# Autodesk Inventor assembly: Humidifier Assembly
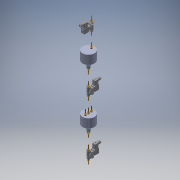
[picture p0: Inventor's stored thumbnail of the model, 180x180]
Saved by Autodesk Inventor 2018 (Build 220112000, 112)
## iProperties
Created: 2020-03-31
Part Number: Humidifier Assembly
Description: STEP AP214
Document SubType Name: Assembly
Designer: emile
Sending System: SolidWorks 2017
Preprocessor: SwSTEP 2.0
Title: Humidifier Assembly.STEP
Revision Number: ANY
## Documents named in this file (5)
- C:\Users\emile\OneDrive\Documents\GitHub\VentilatorCovid19\Respirator\MultiLine\Humidificator\Humidifier Assembly.iam
- C:\Users\emile\OneDrive\Documents\GitHub\VentilatorCovid19\Respirator\MultiLine\Humidificator\Humidifier Botom Funnel.ipt
- C:\Users\emile\OneDrive\Documents\GitHub\VentilatorCovid19\Respirator\MultiLine\SolenoidValve.iam
- C:\Users\emile\OneDrive\Documents\GitHub\VentilatorCovid19\Respirator\Peep\AirPressure\Brass Barbed Hose Fitting for Air and Water.ipt
- C:\Users\emile\OneDrive\Documents\GitHub\VentilatorCovid19\Respirator\MultiLine\Humidificator\HumidifierTopFunnel.ipt
## Components (11 placed, 4 different names)
1. Humidifier Botom Funnel_1 — Mate:1, Mate:2, Mate:11, Mate:12, Mate:15
2. Humidifier Botom Funnel_2 — Mate:5, Mate:6, Mate:7, Mate:8, Mate:9, Mate:10, Mate:13, Mate:14, Mate:15
3. SolenoidValve:1 [sub-assembly] — Mate:17, Angle:1, Mate:18, Mate:19, Flush:1
4. SolenoidValve:2 [sub-assembly] — Mate:20, Angle:2
5. Brass Barbed Hose Fitting for Air and Water:1 — Mate:1, Mate:2, Mate:16, Mate:20
6. Brass Barbed Hose Fitting for Air and Water:4 — Mate:6, Mate:9, Mate:18
7. Brass Barbed Hose Fitting for Air and Water:5 — Mate:5, Mate:8, Mate:16
8. Brass Barbed Hose Fitting for Air and Water:6 — Mate:7, Mate:10
9. Brass Barbed Hose Fitting for Air and Water:7 — Mate:13, Mate:14, Mate:21, Mate:22
10. Brass Barbed Hose Fitting for Air and Water:8 — Mate:11, Mate:12, Mate:17, Mate:19
11. SolenoidValve:3 [sub-assembly] — Mate:21, Mate:22, Flush:1
## Relationships (23: Mate 20, Angle 2, Flush 1)
- Mate:1: Humidifier Botom Funnel_1 ↔ Brass Barbed Hose Fitting for Air and Water:1
- Mate:2: Humidifier Botom Funnel_1 ↔ Brass Barbed Hose Fitting for Air and Water:1
- Mate:5: Humidifier Botom Funnel_2 ↔ Brass Barbed Hose Fitting for Air and Water:5
- Mate:6: Humidifier Botom Funnel_2 ↔ Brass Barbed Hose Fitting for Air and Water:4
- Mate:7: Humidifier Botom Funnel_2 ↔ Brass Barbed Hose Fitting for Air and Water:6
- Mate:8: Humidifier Botom Funnel_2 ↔ Brass Barbed Hose Fitting for Air and Water:5
- Mate:9: Humidifier Botom Funnel_2 ↔ Brass Barbed Hose Fitting for Air and Water:4
- Mate:10: Humidifier Botom Funnel_2 ↔ Brass Barbed Hose Fitting for Air and Water:6
- Mate:11: Humidifier Botom Funnel_1 ↔ Brass Barbed Hose Fitting for Air and Water:8
- Mate:12: Humidifier Botom Funnel_1 ↔ Brass Barbed Hose Fitting for Air and Water:8
- Mate:13: Humidifier Botom Funnel_2 ↔ Brass Barbed Hose Fitting for Air and Water:7
- Mate:14: Humidifier Botom Funnel_2 ↔ Brass Barbed Hose Fitting for Air and Water:7
- Mate:15: Humidifier Botom Funnel_1 ↔ Humidifier Botom Funnel_2
- Mate:16: Brass Barbed Hose Fitting for Air and Water:1 ↔ Brass Barbed Hose Fitting for Air and Water:5
- Mate:17: SolenoidValve:1 ↔ Brass Barbed Hose Fitting for Air and Water:8
- Angle:1 (0 deg): SolenoidValve:1
- Mate:18 (50.8 mm): SolenoidValve:1 ↔ Brass Barbed Hose Fitting for Air and Water:4
- Mate:19 (50.8 mm): SolenoidValve:1 ↔ Brass Barbed Hose Fitting for Air and Water:8
- Mate:20: SolenoidValve:2 ↔ Brass Barbed Hose Fitting for Air and Water:1
- Angle:2 (180 deg): SolenoidValve:2
- Mate:21: Brass Barbed Hose Fitting for Air and Water:7 ↔ SolenoidValve:3
- Mate:22 (50.8 mm): Brass Barbed Hose Fitting for Air and Water:7 ↔ SolenoidValve:3
- Flush:1: SolenoidValve:1 ↔ SolenoidValve:3
